# Autodesk Inventor assembly: Frame End
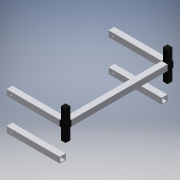
[picture p0: Inventor's stored thumbnail of the model, 180x180]
Saved by Autodesk Inventor 2017 (Build 210142000, 142)
## iProperties
Created: 2019-12-06
Part Number: Frame End
Document SubType Name: Assembly
Designer: S346553810
Author: S346553810
## Documents named in this file (4)
- \\ad.ocdsb.ca\studenthome\3\S338674153\FRC 2020\FullRobotRefactor\SubFrame\Frame End.iam
- \\ad.ocdsb.ca\studenthome\3\S338674153\FRC 2020\FullRobotRefactor\SubFrame\End cross-member.iam
- \\ad.ocdsb.ca\studenthome\3\S338674153\FRC 2020\FullRobotRefactor\SubFrame\1in sq tub - 10-875.ipt
- \\ad.ocdsb.ca\studenthome\3\S338674153\FRC 2020\FullRobotRefactor\SubFrame\End cross-member top.iam
## Components (6 placed, 3 different names)
1. End cross-member:2 [sub-assembly]
2. 1in sq tub - 10-875:1 — Flush:13, Flush:14, Mate:5
3. 1in sq tub - 10-875:2 — Mate:2, Mate:3, Flush:10, Flush:13, Flush:14, Mate:5
4. 1in sq tub - 10-875:3 — Flush:11, Flush:12, Mate:4
5. 1in sq tub - 10-875:4 — Mate:1, Flush:1, Flush:2, Flush:11, Flush:12, Mate:4
6. End cross-member top:1 [sub-assembly] — Mate:1, Flush:1, Flush:2, Mate:2, Mate:3, Flush:10
## Relationships (12: Flush 7, Mate 5)
- Mate:1: 1in sq tub - 10-875:4 ↔ End cross-member top:1
- Flush:1: 1in sq tub - 10-875:4 ↔ End cross-member top:1
- Flush:2: 1in sq tub - 10-875:4 ↔ End cross-member top:1
- Mate:2: 1in sq tub - 10-875:2 ↔ End cross-member top:1
- Mate:3: 1in sq tub - 10-875:2 ↔ End cross-member top:1
- Flush:10: 1in sq tub - 10-875:2 ↔ End cross-member top:1
- Flush:11: 1in sq tub - 10-875:3 ↔ 1in sq tub - 10-875:4
- Flush:12: 1in sq tub - 10-875:3 ↔ 1in sq tub - 10-875:4
- Mate:4 (114.3 mm): 1in sq tub - 10-875:3 ↔ 1in sq tub - 10-875:4
- Flush:13: 1in sq tub - 10-875:1 ↔ 1in sq tub - 10-875:2
- Flush:14: 1in sq tub - 10-875:1 ↔ 1in sq tub - 10-875:2
- Mate:5 (114.3 mm): 1in sq tub - 10-875:1 ↔ 1in sq tub - 10-875:2
